# Autodesk Inventor assembly: am-0144a SmoothGrip Wheel
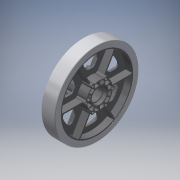
[picture p0: Inventor's stored thumbnail of the model, 180x180]
Saved by Autodesk Inventor 2019 (Build 230136000, 136)
## iProperties
Created: 2018-12-06
Part Number: am-0144a SmoothGrip Wheel
Description: STEP AP214
Document SubType Name: Assembly
Designer: Michael Olukoya
Sending System: SolidWorks 2018
Preprocessor: SwSTEP 2.0
Title: am-0144a SmoothGrip Wheel.STEP
Revision Number: ANY
## Documents named in this file (3)
- C:\Users\Michael Olukoya\Desktop\Turtle BOT- AI\New Bot components\am-0144a SmoothGrip Wheel.iam
- C:\Users\Michael Olukoya\Desktop\Turtle BOT- AI\New Bot components\6 wheel Rev 4.ipt
- C:\Users\Michael Olukoya\Desktop\Turtle BOT- AI\New Bot components\SmoothGrip Tread.ipt
## Components (2 placed, 2 different names)
1. 6 wheel Rev 4_1 — Flush:1, Rotational:1
2. SmoothGrip Tread_2 — Flush:1, Rotational:1
## Relationships (2: Flush 1, RevoluteJoint 1)
- Flush:1: 6 wheel Rev 4_1 ↔ SmoothGrip Tread_2
- Rotational:1 [RevoluteJoint]: 6 wheel Rev 4_1 ↔ SmoothGrip Tread_2
